# Autodesk Inventor assembly: 前足
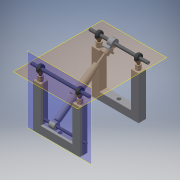
[picture p0: Inventor's stored thumbnail of the model, 180x180]
Saved by Autodesk Inventor 2018 (Build 220112000, 112)
## iProperties
Created: 2017-09-13
Part Number: 前足
Material: 一般
Document SubType Name: Assembly
Designer: mura5
Author: mura5
## Documents named in this file (7)
- C:\Users\mura5\Documents\RBBR\cart\前足\前足.iam
- C:\Users\mura5\Documents\RBBR\cart\前足\Aアーム下.iam
- C:\Users\mura5\Documents\RBBR\cart\iko_POS_12\AIS2014\POS 12.iam
- C:\Users\mura5\Documents\RBBR\cart\前足\軸.ipt
- C:\Users\mura5\Documents\RBBR\cart\スプリング\スプリング.iam
- C:\Users\mura5\Documents\RBBR\cart\前足\軸10mm.ipt
- C:\Users\mura5\Documents\RBBR\cart\前足\Aアーム上.iam
## Components (10 placed, 6 different names)
1. Aアーム上:1 [sub-assembly] — 回転:1, 回転:2
2. Aアーム下:2 [sub-assembly] — 回転:3, 回転:4, 角度:1, 円柱状:5, 角度:2, メイト:3
3. POS 12:1 [sub-assembly] — 回転:1, 円柱状:1
4. POS 12:2 [sub-assembly] — 回転:2, 円柱状:2, フラッシュ:1
5. POS 12:3 [sub-assembly] — 回転:3, 円柱状:4, フラッシュ:3
6. POS 12:4 [sub-assembly] — 回転:4, 円柱状:3
7. 軸:1 — 円柱状:1, 円柱状:2, フラッシュ:1, メイト:1, フラッシュ:2, 正接:1, 回転:5, 円柱状:6
8. 軸:2 — メイト:1, フラッシュ:2, 正接:2, 正接:3, メイト:2, 円柱状:3, 円柱状:4, フラッシュ:3
9. スプリング:1 [sub-assembly] — 回転:5, 回転:7, 円柱状:6, 円柱状:7, メイト:3
10. 軸10mm:1 — 回転:7, 円柱状:5, 円柱状:7
## Relationships (24: CylindricalJoint 7, RevoluteJoint 6, Flush 3, Mate 3, Tangent 3, Angle 2)
- 回転:1 [RevoluteJoint] (10 mm): Aアーム上:1 ↔ POS 12:1
- 回転:2 [RevoluteJoint] (10 mm): Aアーム上:1 ↔ POS 12:2
- 回転:3 [RevoluteJoint] (10 mm): Aアーム下:2 ↔ POS 12:3
- 回転:4 [RevoluteJoint] (10 mm): Aアーム下:2 ↔ POS 12:4
- 円柱状:1 [CylindricalJoint]: POS 12:1 ↔ 軸:1
- 円柱状:2 [CylindricalJoint]: POS 12:2 ↔ 軸:1
- フラッシュ:1 [Flush] (35 mm): POS 12:2 ↔ 軸:1
- メイト:1 [Mate] (250 mm): 軸:1 ↔ 軸:2
- フラッシュ:2 [Flush]: 軸:1 ↔ 軸:2
- 正接:1 [Tangent]: 軸:1
- 正接:2 [Tangent]: 軸:2
- 正接:3 [Tangent]: 軸:2
- メイト:2 [Mate]: 軸:2
- 円柱状:3 [CylindricalJoint]: POS 12:4 ↔ 軸:2
- 円柱状:4 [CylindricalJoint]: POS 12:3 ↔ 軸:2
- フラッシュ:3 [Flush] (35 mm): POS 12:3 ↔ 軸:2
- 回転:5 [RevoluteJoint]: 軸:1 ↔ スプリング:1
- 角度:1 [Angle] (-18 deg): Aアーム下:2
- 回転:7 [RevoluteJoint]: スプリング:1 ↔ 軸10mm:1
- 円柱状:5 [CylindricalJoint]: Aアーム下:2 ↔ 軸10mm:1
- 角度:2 [Angle] (0 deg): Aアーム下:2
- 円柱状:6 [CylindricalJoint]: 軸:1 ↔ スプリング:1
- 円柱状:7 [CylindricalJoint]: スプリング:1 ↔ 軸10mm:1
- メイト:3 [Mate] (30 mm): Aアーム下:2 ↔ スプリング:1
